# Autodesk Inventor assembly: ToolDock
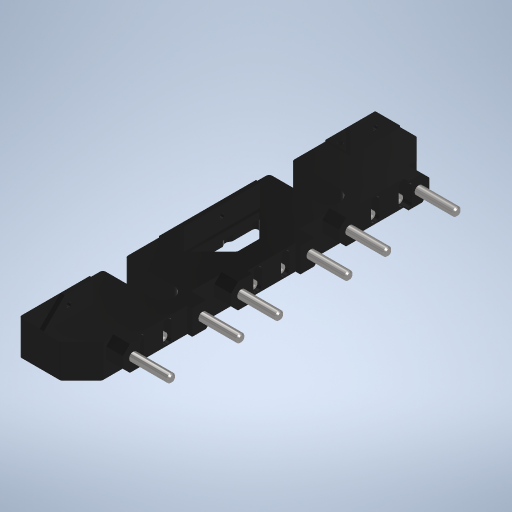
[picture p0: Inventor's stored thumbnail of the model, 512x512]
Saved by Autodesk Inventor 2023.2 (Build 272271000, 271)
## iProperties
Created: 2022-07-04
Part Number: ToolDock
Document SubType Name: Assembly
Designer: Remo
Author: Remo
## Documents named in this file (7)
- C:\Users\remop\OneDrive\Documents\Inventor\3D Printers\LuEVO\Mk4_Toolchanger\ToolDock.iam
- C:\Users\remop\OneDrive\Documents\Inventor\3D Printers\LuEVO\Mk4_Toolchanger\ToolDock_Base.ipt
- C:\Users\remop\OneDrive\Documents\Inventor\3D Printers\LuEVO\Mk4_Toolchanger\ToolDock_Center.ipt
- C:\Users\remop\OneDrive\Documents\Inventor\3D Printers\LuEVO\Mk4_Toolchanger\ToolDock_Left.ipt
- C:\Users\remop\OneDrive\Documents\Inventor\Content Center Files\R2023\en-US\AS 1420\AS 1420 - 1973 - M3 x 16.ipt
- C:\Users\remop\OneDrive\Documents\Inventor\3D Printers\LuEVO\Mk4_Toolchanger\ToolDock_Bolt.ipt
- C:\Users\remop\OneDrive\Documents\Inventor\3D Printers\LuEVO\Mk4_Toolchanger\ToolDock_R.ipt
## Components (16 placed, 6 different names)
1. ToolDock_Base:1 — Mate:1, Mate:2, Mate:3, Mate:4, Mate:5, Mate:6, Rigid:5
2. ToolDock_Center:1 — Mate:1, Mate:3, Mate:5, Insert:4, Insert:7, Rigid:1, Rigid:2
3. ToolDock_Left:1 — Mate:2, Mate:4, Mate:6, Insert:1, Insert:3, Rigid:3, Rigid:4
4. ToolDock_R:1 — Rigid:5, Rotational:1, Rotational:2
5. AS 1420 - Metric M3 x 16:1 — Insert:1
6. AS 1420 - Metric M3 x 16:3 — Insert:3
7. AS 1420 - Metric M3 x 16:4 — Insert:4
8. AS 1420 - Metric M3 x 16:7 — Insert:7
9. ToolDock_Bolt:1 — Rigid:3
10. ToolDock_Bolt:2 — Rigid:1
11. ToolDock_Bolt:3 — Rigid:4
12. ToolDock_Bolt:4 — Rigid:2
13. ToolDock_Bolt:5 — Rotational:2
14. ToolDock_Bolt:6 — Rotational:1
15. AS 1420 - Metric M3 x 16:10
16. AS 1420 - Metric M3 x 16:11
## Relationships (17: Mate 6, WeldJoint 5, Insert 4, RevoluteJoint 2)
- Mate:1: ToolDock_Base:1 ↔ ToolDock_Center:1
- Mate:2: ToolDock_Base:1 ↔ ToolDock_Left:1
- Mate:3: ToolDock_Base:1 ↔ ToolDock_Center:1
- Mate:4: ToolDock_Base:1 ↔ ToolDock_Left:1
- Mate:5: ToolDock_Base:1 ↔ ToolDock_Center:1
- Mate:6: ToolDock_Base:1 ↔ ToolDock_Left:1
- Insert:1: ToolDock_Left:1 ↔ AS 1420 - Metric M3 x 16:1
- Insert:3: ToolDock_Left:1 ↔ AS 1420 - Metric M3 x 16:3
- Insert:4: ToolDock_Center:1 ↔ AS 1420 - Metric M3 x 16:4
- Insert:7: ToolDock_Center:1 ↔ AS 1420 - Metric M3 x 16:7
- Rigid:1 [WeldJoint]: ToolDock_Center:1 ↔ ToolDock_Bolt:2
- Rigid:2 [WeldJoint]: ToolDock_Center:1 ↔ ToolDock_Bolt:4
- Rigid:3 [WeldJoint]: ToolDock_Left:1 ↔ ToolDock_Bolt:1
- Rigid:4 [WeldJoint]: ToolDock_Left:1 ↔ ToolDock_Bolt:3
- Rigid:5 [WeldJoint]: ToolDock_Base:1 ↔ ToolDock_R:1
- Rotational:1 [RevoluteJoint]: ToolDock_R:1 ↔ ToolDock_Bolt:6
- Rotational:2 [RevoluteJoint]: ToolDock_R:1 ↔ ToolDock_Bolt:5
